# Autodesk Inventor assembly: 8 inch mecanum with toughbox (left)
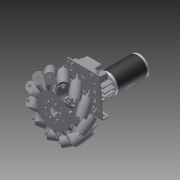
[picture p0: Inventor's stored thumbnail of the model, 180x180]
Saved by Autodesk Inventor 2014 (Build 180170000, 170)
## iProperties
Created: 2015-01-10
Part Number: 8 inch mecanum with toughbox (left)
Document SubType Name: Assembly
Designer: student
Author: student
## Documents named in this file (6)
- C:\Users\student\Documents\Inventor\2015 Recycle Rush\8 inch mecanum with toughbox (left).iam
- C:\Users\student\Documents\Inventor\2015 Recycle Rush\am-0077a-500 Key Hub r2_MIR1.ipt
- C:\Users\student\Documents\Inventor\2015 Recycle Rush\Derived Toughbox mini.ipt
- C:\Users\student\Documents\Inventor\Dillon And Justin\Imported Components\MOT_CIM-Motor_217-2000.iam\MOT_CIM-Motor_217-2000.iam.iam
- C:\Users\student\Documents\Inventor\2015 Recycle Rush\Derived Left Mecanum_MIR.ipt
- MOT_CIM-Motor_217-2000.iam
## Components (4 placed, 4 different names)
1. am-0077a-500 Key Hub r2_MIR1:2 — Mate:4, Angle:1, Mate:7, Mate:8, Mate:9
2. Derived Toughbox mini:1 — Mate:4, Mate:10, Mate:11
3. MOT_CIM-Motor_217-2000.iam:1 [sub-assembly] — Mate:10, Mate:11
4. Derived Left Mecanum_MIR:1 — Angle:1, Mate:7, Mate:8, Mate:9
## Relationships (7: Mate 6, Angle 1)
- Mate:4: am-0077a-500 Key Hub r2_MIR1:2 ↔ Derived Toughbox mini:1
- Angle:1 (0 deg): am-0077a-500 Key Hub r2_MIR1:2 ↔ Derived Left Mecanum_MIR:1
- Mate:7: am-0077a-500 Key Hub r2_MIR1:2 ↔ Derived Left Mecanum_MIR:1
- Mate:8: am-0077a-500 Key Hub r2_MIR1:2 ↔ Derived Left Mecanum_MIR:1
- Mate:9: am-0077a-500 Key Hub r2_MIR1:2 ↔ Derived Left Mecanum_MIR:1
- Mate:10: Derived Toughbox mini:1 ↔ MOT_CIM-Motor_217-2000.iam:1
- Mate:11: Derived Toughbox mini:1 ↔ MOT_CIM-Motor_217-2000.iam:1
